# Autodesk Inventor assembly: micheals magic rod
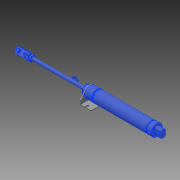
[picture p0: Inventor's stored thumbnail of the model, 180x180]
Saved by Autodesk Inventor 2013 (Build 170138000, 138)
## iProperties
Created: 2013-03-16
Part Number: micheals magic rod
Document SubType Name: Assembly
Designer: Arpan
Author: Arpan
## Documents named in this file (3)
- C:\Users\Arpan\Documents\GitHub\frc2013CAD\micheals magic rod.iam
- C:\Users\Arpan\Documents\GitHub\frc2013CAD\Ninja cylinder thing.iam
- C:\Users\Arpan\Documents\GitHub\frc2013CAD\ninja cylinder foot bracket.ipt
## Components (2 placed, 2 different names)
1. Ninja cylinder thing:1 [sub-assembly] — Mate:1, Angle:1, Angle:2, Mate:2
2. ninja cylinder foot bracket:1 — Mate:1, Angle:1, Angle:2, Mate:2
## Relationships (4: Mate 2, Angle 2)
- Mate:1: Ninja cylinder thing:1 ↔ ninja cylinder foot bracket:1
- Angle:1 (180 deg): Ninja cylinder thing:1 ↔ ninja cylinder foot bracket:1
- Angle:2 (0 deg): Ninja cylinder thing:1 ↔ ninja cylinder foot bracket:1
- Mate:2: Ninja cylinder thing:1 ↔ ninja cylinder foot bracket:1
